# Autodesk Inventor assembly: PlanB
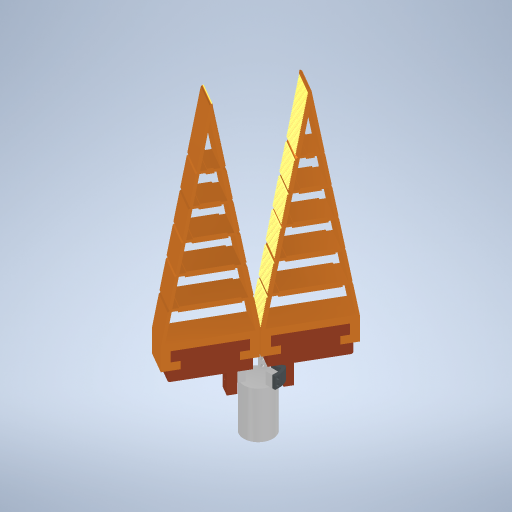
[picture p0: Inventor's stored thumbnail of the model, 512x512]
Saved by Autodesk Inventor 2024 (Build 280153000, 153)
## iProperties
Created: 2023-12-04
Part Number: PlanB
Document SubType Name: Assembly
Designer: Juan_Daleman
Author: Juan_Daleman
## Documents named in this file (5)
- D:\Documentos\Proyectos_U\Semestre 9\Robotica\Proyecto\PlanB.iam
- D:\Documentos\Proyectos_U\Semestre 9\Robotica\Proyecto\Dedo Gripper.ipt
- D:\Documentos\Proyectos_U\Semestre 9\Robotica\Proyecto\Basegripper.ipt
- D:\Documentos\Proyectos_U\Semestre 9\Robotica\Proyecto\acople.ipt
- D:\Documentos\Proyectos_U\Semestre 9\Robotica\Proyecto\Cilindro.ipt
## Components (6 placed, 4 different names)
1. Dedo Gripper:1 — Mate:1, Mate:2, Flush:1, Flush:3
2. Dedo Gripper:2 — Mate:3, Mate:4, Flush:2, Flush:3
3. Basegripper:1 — Mate:1, Mate:2, Flush:1, Insert:6
4. Basegripper:2 — Mate:3, Mate:4, Flush:2, Insert:5, Mate:5
5. acople:1 — Insert:4, Insert:6
6. Cilindro:1 — Insert:4, Insert:5, Mate:5, Flush:4, Flush:5
## Relationships (13: Mate 5, Flush 5, Insert 3)
- Mate:1: Dedo Gripper:1 ↔ Basegripper:1
- Mate:2: Dedo Gripper:1 ↔ Basegripper:1
- Flush:1: Dedo Gripper:1 ↔ Basegripper:1
- Mate:3: Dedo Gripper:2 ↔ Basegripper:2
- Mate:4: Dedo Gripper:2 ↔ Basegripper:2
- Flush:2: Dedo Gripper:2 ↔ Basegripper:2
- Flush:3: Dedo Gripper:1 ↔ Dedo Gripper:2
- Insert:4: acople:1 ↔ Cilindro:1
- Insert:5: Basegripper:2 ↔ Cilindro:1
- Mate:5: Basegripper:2 ↔ Cilindro:1
- Insert:6: Basegripper:1 ↔ acople:1
- Flush:4: Cilindro:1
- Flush:5: Cilindro:1
